# Autodesk Inventor assembly: Plow Part
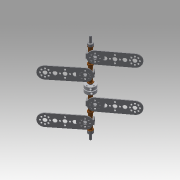
[picture p0: Inventor's stored thumbnail of the model, 180x180]
Saved by Autodesk Inventor 2016 (Build 200138000, 138)
## iProperties
Created: 2015-10-31
Part Number: Plow Part
Document SubType Name: Assembly
Designer: RoboticsUser
Author: RoboticsUser
## Documents named in this file (9)
- C:\Robotics\CAD\2015-16\custom cad parts\Plow Part.iam
- C:\Robotics\CAD\2015-16\COTSParts\Tetrix\Tetrix shaft 100mm.ipt
- C:\Robotics\CAD\2015-16\COTSParts\Tetrix\Bronze bushing.ipt
- C:\Robotics\CAD\2015-16\COTSParts\Tetrix\Tetrix Lego Adapter.ipt
- C:\Robotics\CAD\2015-16\COTSParts\Tetrix\Tetrix shaft collar.ipt
- C:\Robotics\CAD\2015-16\COTSParts\Tetrix\Tetrix Hub - axle_MIR.ipt
- C:\Users\RoboticsUser\Desktop\2015-16 CAD\custom cad parts\Flap Plow.ipt
- C:\Users\RoboticsUser\Desktop\2015-16 CAD\COTSParts\Tetrix\Tetrix bracket - flat.ipt
- C:\Robotics\CAD\2015-16\COTSParts\Tetrix\Pitsco Education-739273.ipt
## Components (26 placed, 8 different names)
1. Tetrix shaft 100mm:1 — Insert:1, Mate:1
2. Bronze bushing:1 — Insert:4, Insert:5
3. Bronze bushing:2 — Insert:9, Insert:10
4. Bronze bushing:4 — Insert:6, Insert:7
5. Bronze bushing:7 — Mate:1, Mate:2, Insert:11
6. Bronze bushing:8 — Insert:7, Insert:8
7. Tetrix shaft 100mm:2 — Insert:2
8. Tetrix Lego Adapter:1 — Insert:8, Insert:9, Insert:22, Insert:23, Insert:25, Mate:5
9. Tetrix Lego Adapter:3 — Insert:5, Insert:6, Insert:21, Mate:3
10. Tetrix Lego Adapter:4 — Insert:11, Insert:12, Insert:19, Insert:20, Insert:24, Mate:4
11. Tetrix shaft collar:2 — Insert:10
12. Tetrix Hub - axle_MIR:1 — Insert:1, Mate:2, Insert:3
13. Tetrix Hub - axle_MIR:2 — Insert:2, Insert:3, Insert:4
14. Bronze bushing:9 — Insert:13, Insert:14
15. Tetrix Lego Adapter:5 — Insert:14, Insert:15, Insert:17, Insert:18
16. Tetrix shaft collar:3 — Insert:16
17. Bronze bushing:12 — Insert:12, Insert:13
18. Bronze bushing:13 — Insert:15, Insert:16
19. Flap Plow:1
20. Flap Plow:2
21. Tetrix bracket - flat:1 — Insert:19, Insert:20
22. Tetrix bracket - flat:2 — Insert:22, Insert:23
23. Pitsco Education-739273:1 — Insert:17, Insert:18
24. Pitsco Education-739273:2 — Insert:21, Mate:3
25. Pitsco Education-739273:3 — Insert:25, Mate:5
26. Pitsco Education-739273:4 — Insert:24, Mate:4
## Relationships (30: Insert 25, Mate 5)
- Insert:1: Tetrix shaft 100mm:1 ↔ Tetrix Hub - axle_MIR:1
- Insert:2: Tetrix shaft 100mm:2 ↔ Tetrix Hub - axle_MIR:2
- Mate:1: Tetrix shaft 100mm:1 ↔ Bronze bushing:7
- Mate:2: Bronze bushing:7 ↔ Tetrix Hub - axle_MIR:1
- Insert:3 (2.032 mm): Tetrix Hub - axle_MIR:1 ↔ Tetrix Hub - axle_MIR:2
- Insert:4: Bronze bushing:1 ↔ Tetrix Hub - axle_MIR:2
- Insert:5: Bronze bushing:1 ↔ Tetrix Lego Adapter:3
- Insert:6: Bronze bushing:4 ↔ Tetrix Lego Adapter:3
- Insert:7: Bronze bushing:4 ↔ Bronze bushing:8
- Insert:8: Bronze bushing:8 ↔ Tetrix Lego Adapter:1
- Insert:9: Bronze bushing:2 ↔ Tetrix Lego Adapter:1
- Insert:10: Bronze bushing:2 ↔ Tetrix shaft collar:2
- Insert:11: Bronze bushing:7 ↔ Tetrix Lego Adapter:4
- Insert:12: Tetrix Lego Adapter:4 ↔ Bronze bushing:12
- Insert:13: Bronze bushing:9 ↔ Bronze bushing:12
- Insert:14: Bronze bushing:9 ↔ Tetrix Lego Adapter:5
- Insert:15: Tetrix Lego Adapter:5 ↔ Bronze bushing:13
- Insert:16: Tetrix shaft collar:3 ↔ Bronze bushing:13
- Insert:17: Tetrix Lego Adapter:5 ↔ Pitsco Education-739273:1
- Insert:18: Tetrix Lego Adapter:5 ↔ Pitsco Education-739273:1
- Insert:19: Tetrix Lego Adapter:4 ↔ Tetrix bracket - flat:1
- Insert:20: Tetrix Lego Adapter:4 ↔ Tetrix bracket - flat:1
- Insert:21: Tetrix Lego Adapter:3 ↔ Pitsco Education-739273:2
- Insert:22: Tetrix Lego Adapter:1 ↔ Tetrix bracket - flat:2
- Insert:23: Tetrix Lego Adapter:1 ↔ Tetrix bracket - flat:2
- Mate:3: Tetrix Lego Adapter:3 ↔ Pitsco Education-739273:2
- Insert:24: Tetrix Lego Adapter:4 ↔ Pitsco Education-739273:4
- Mate:4: Tetrix Lego Adapter:4 ↔ Pitsco Education-739273:4
- Insert:25: Tetrix Lego Adapter:1 ↔ Pitsco Education-739273:3
- Mate:5: Tetrix Lego Adapter:1 ↔ Pitsco Education-739273:3
